# Autodesk Inventor assembly: Lopez_Tripod
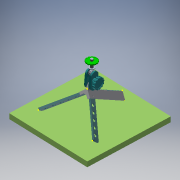
[picture p0: Inventor's stored thumbnail of the model, 180x180]
Saved by Autodesk Inventor 2018 (Build 220112000, 112)
## iProperties
Created: 2018-02-23
Part Number: Lopez_Tripod
Document SubType Name: Assembly
Designer: clopez06
Mass: 25.6819 g
Surface Area: 240.693 cm^2
Volume: 26.944 cm^3
Density: 0.953159 g/cm^3
Author: clopez06
## Documents named in this file (10)
- J:\ES18\Lopez_ES18_Tripod\Lopez_Tripod.iam
- J:\ES18\Lopez_ES18_Tripod\Lopez_CenterLeg.ipt
- J:\ES18\Lopez_ES18_Tripod\Lopez_LeftLeg.ipt
- J:\ES18\Lopez_ES18_Tripod\Lopez_RigthLeg.ipt
- J:\ES18\Lopez_ES18_Tripod\Lopez_LeftClamp.ipt
- J:\ES18\Lopez_ES18_Tripod\Tripod_BallShaft.ipt
- J:\ES18\Lopez_ES18_Tripod\Lopez_RightClamp.ipt
- J:\ES18\Lopez_ES18_Tripod\Lopez_Knob.ipt
- J:\ES18\Lopez_ES18_Tripod\Tripod_Wheel.ipt
- J:\ES18\Lopez_ES18_Tripod\Tripod_Table.ipt
## Components (9 placed, 9 different names)
1. Lopez_CenterLeg:1 — Mate:3, Mate:4, Insert:1, Insert:2, Insert:3, Angle:1, Angle:2, Mate:11
2. Lopez_RigthLeg:1 — Mate:3, Mate:4, Angle:2, Angle:4
3. Lopez_LeftLeg:1 — Insert:1, Angle:1, Angle:3
4. Lopez_LeftClamp:1 — Mate:5, Insert:3
5. Tripod_BallShaft:1 — Mate:5, Mate:6, Mate:7, Angle:5
6. Lopez_RightClamp:1 — Insert:2, Mate:6, Insert:4
7. Lopez_Knob:1 — Insert:4
8. Tripod_Wheel:1 — Mate:7
9. Tripod_Table:1 — Mate:11, Mate:12, Angle:3, Angle:4, Angle:5
## Relationships (16: Mate 7, Angle 5, Insert 4)
- Mate:3: Lopez_CenterLeg:1 ↔ Lopez_RigthLeg:1
- Mate:4: Lopez_CenterLeg:1 ↔ Lopez_RigthLeg:1
- Insert:1: Lopez_CenterLeg:1 ↔ Lopez_LeftLeg:1
- Mate:5: Lopez_LeftClamp:1 ↔ Tripod_BallShaft:1
- Insert:2: Lopez_CenterLeg:1 ↔ Lopez_RightClamp:1
- Insert:3: Lopez_CenterLeg:1 ↔ Lopez_LeftClamp:1
- Mate:6: Tripod_BallShaft:1 ↔ Lopez_RightClamp:1
- Insert:4: Lopez_RightClamp:1 ↔ Lopez_Knob:1
- Mate:7: Tripod_BallShaft:1 ↔ Tripod_Wheel:1
- Angle:1 (106.87 deg): Lopez_CenterLeg:1 ↔ Lopez_LeftLeg:1
- Angle:2 (106.87 deg): Lopez_CenterLeg:1 ↔ Lopez_RigthLeg:1
- Mate:11: Lopez_CenterLeg:1 ↔ Tripod_Table:1
- Mate:12: Tripod_Table:1
- Angle:3 (116.88 deg): Lopez_LeftLeg:1 ↔ Tripod_Table:1
- Angle:4 (116.88 deg): Lopez_RigthLeg:1 ↔ Tripod_Table:1
- Angle:5 (0 deg): Tripod_BallShaft:1 ↔ Tripod_Table:1
